# Autodesk Inventor assembly: 付け根_1
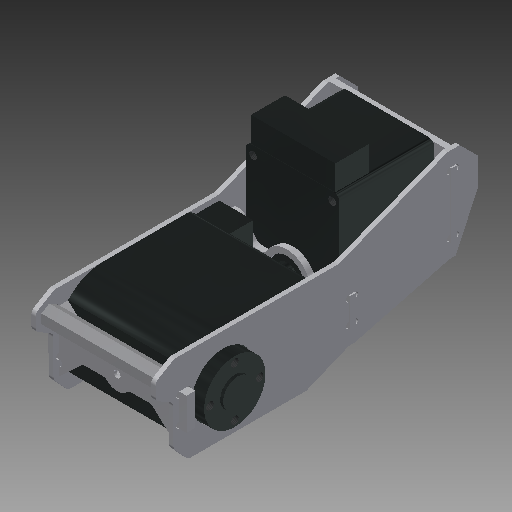
[picture p0: Inventor's stored thumbnail of the model, 512x512]
Saved by Autodesk Inventor 2018 (Build 220112000, 112)
## iProperties
Created: 2016-04-27
Part Number: 付け根_1
Document SubType Name: Assembly
Designer: hiroaki
Mass: 228.077 g
Surface Area: 379.105 cm^2
Volume: 115.513 cm^3
Density: 1.97447 g/cm^3
Author: hiroaki
## Documents named in this file (9)
- Z:\OPR\OpenPlatform_ver1_0\下半身\足首\足首_1.iam
- Z:\OPR\OpenPlatform_ver1_0\既製品\B3M11xx.ipt
- Z:\OPR\OpenPlatform_ver1_0\下半身\足首\足首_メインフレーム_1_1.ipt
- Z:\OPR\OpenPlatform_ver1_0\下半身\足首\足首_サブフレーム_1_1.ipt
- Z:\OPR\OpenPlatform_ver1_0\下半身\足首\足首_サブフレーム_1_2.ipt
- Z:\OPR\OpenPlatform_ver1_0\下半身\足首\足首_メインフレーム_1_1_MIR.ipt
- Z:\OPR\OpenPlatform_ver1_0\下半身\足首\足首_サブフレーム_1_3.ipt
- Z:\OPR\OpenPlatform_ver1_0\既製品\B3M10xx.ipt
- Z:\OPR\OpenPlatform_ver1_0\既製品\ASU-340.ipt
## Components (9 placed, 7 different names)
1. B3M11xx:1 — 挿入:24, 挿入:25, 挿入:26, 挿入:27, 挿入:36, 挿入:37, 挿入:38, 挿入:39, メイト:7
2. 足首_メインフレーム_1_1:1 — 挿入:24, 挿入:25, 挿入:26, 挿入:27, メイト:1, メイト:2, メイト:3, メイト:4, メイト:5, メイト:6, メイト:8, 挿入:46, 挿入:48, 角度:2
3. 足首_サブフレーム_1_1:1 — メイト:1, メイト:2, メイト:3, 挿入:42, 挿入:45
4. 足首_サブフレーム_1_2:1 — メイト:4, メイト:5, メイト:6, 挿入:43, 挿入:44
5. 足首_メインフレーム_1_1_MIR:1 — 挿入:36, 挿入:37, 挿入:38, 挿入:39, メイト:9, 挿入:47, 挿入:49, 角度:1
6. 足首_サブフレーム_1_3:1 — メイト:7, メイト:8, メイト:9
7. B3M11xx:3 — 挿入:42, 挿入:43, 挿入:44, 挿入:45
8. ASU-340:1 — 挿入:46, 挿入:47, 角度:1
9. ASU-340:2 — 挿入:48, 挿入:49, 角度:2
## Relationships (27: Insert 16, Mate 9, Angle 2)
- 挿入:24 [Insert]: B3M11xx:1 ↔ 足首_メインフレーム_1_1:1
- 挿入:25 [Insert]: B3M11xx:1 ↔ 足首_メインフレーム_1_1:1
- 挿入:26 [Insert]: B3M11xx:1 ↔ 足首_メインフレーム_1_1:1
- 挿入:27 [Insert]: B3M11xx:1 ↔ 足首_メインフレーム_1_1:1
- メイト:1 [Mate] (0.025 mm): 足首_メインフレーム_1_1:1 ↔ 足首_サブフレーム_1_1:1
- メイト:2 [Mate]: 足首_メインフレーム_1_1:1 ↔ 足首_サブフレーム_1_1:1
- メイト:3 [Mate] (0.025 mm): 足首_メインフレーム_1_1:1 ↔ 足首_サブフレーム_1_1:1
- メイト:4 [Mate]: 足首_メインフレーム_1_1:1 ↔ 足首_サブフレーム_1_2:1
- メイト:5 [Mate] (0.025 mm): 足首_メインフレーム_1_1:1 ↔ 足首_サブフレーム_1_2:1
- メイト:6 [Mate] (0.025 mm): 足首_メインフレーム_1_1:1 ↔ 足首_サブフレーム_1_2:1
- 挿入:36 [Insert]: B3M11xx:1 ↔ 足首_メインフレーム_1_1_MIR:1
- 挿入:37 [Insert]: B3M11xx:1 ↔ 足首_メインフレーム_1_1_MIR:1
- 挿入:38 [Insert]: B3M11xx:1 ↔ 足首_メインフレーム_1_1_MIR:1
- 挿入:39 [Insert]: B3M11xx:1 ↔ 足首_メインフレーム_1_1_MIR:1
- メイト:7 [Mate]: B3M11xx:1 ↔ 足首_サブフレーム_1_3:1
- メイト:8 [Mate]: 足首_メインフレーム_1_1:1 ↔ 足首_サブフレーム_1_3:1
- メイト:9 [Mate] (0.025 mm): 足首_メインフレーム_1_1_MIR:1 ↔ 足首_サブフレーム_1_3:1
- 挿入:42 [Insert]: 足首_サブフレーム_1_1:1 ↔ B3M11xx:3
- 挿入:43 [Insert]: 足首_サブフレーム_1_2:1 ↔ B3M11xx:3
- 挿入:44 [Insert]: 足首_サブフレーム_1_2:1 ↔ B3M11xx:3
- 挿入:45 [Insert]: 足首_サブフレーム_1_1:1 ↔ B3M11xx:3
- 挿入:46 [Insert]: 足首_メインフレーム_1_1:1 ↔ ASU-340:1
- 挿入:47 [Insert]: 足首_メインフレーム_1_1_MIR:1 ↔ ASU-340:1
- 挿入:48 [Insert]: 足首_メインフレーム_1_1:1 ↔ ASU-340:2
- 挿入:49 [Insert]: 足首_メインフレーム_1_1_MIR:1 ↔ ASU-340:2
- 角度:1 [Angle] (0 deg): 足首_メインフレーム_1_1_MIR:1 ↔ ASU-340:1
- 角度:2 [Angle] (0 deg): 足首_メインフレーム_1_1:1 ↔ ASU-340:2
